# Autodesk Inventor assembly: zitvlak
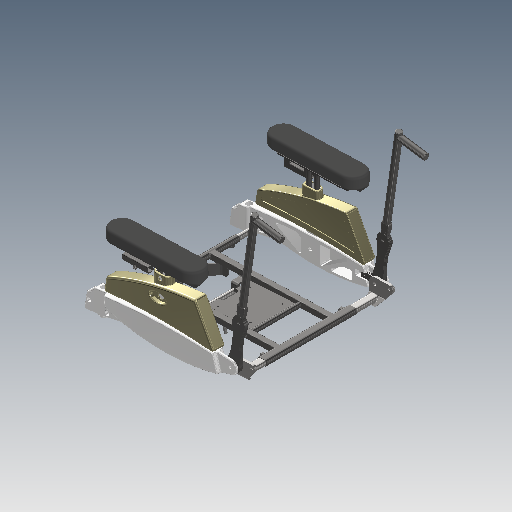
[picture p0: Inventor's stored thumbnail of the model, 512x512]
Saved by Autodesk Inventor 2020.3 (Build 243373000, 373)
## iProperties
Created: 2020-09-15
Part Number: zitvlak
Document SubType Name: Assembly
Designer: Svend
Author: Svend
## Documents named in this file (14)
- C:\Users\Svend\OneDrive\Documents\GitHub\Rolstoel\zitvlak.iam
- C:\Users\Svend\OneDrive\Documents\GitHub\Rolstoel\buis 18 mm.ipt
- C:\Users\Svend\OneDrive\Documents\GitHub\Rolstoel\frame achterkant links.ipt
- C:\Users\Svend\OneDrive\Documents\GitHub\Rolstoel\frame achterkant.ipt
- C:\Users\Svend\OneDrive\Documents\GitHub\Rolstoel\frame zitvlak.ipt
- C:\Users\Svend\OneDrive\Documents\GitHub\Rolstoel\scharnier.iam
- C:\Users\Svend\OneDrive\Documents\GitHub\Rolstoel\stelbuis.ipt
- C:\Users\Svend\OneDrive\Documents\GitHub\Rolstoel\lift connectie.ipt
- C:\Users\Svend\OneDrive\Documents\GitHub\Rolstoel\stelblokje.ipt
- C:\Users\Svend\OneDrive\Documents\GitHub\Rolstoel\zijkant.ipt
- C:\Users\Svend\OneDrive\Documents\GitHub\Rolstoel\armsteun links.iam
- C:\Users\Svend\OneDrive\Documents\GitHub\Rolstoel\zijkant rechts.ipt
- C:\Users\Svend\OneDrive\Documents\GitHub\Rolstoel\armsteun rechts.iam
- C:\Users\Svend\OneDrive\Documents\GitHub\Rolstoel\handvaten.ipt
## Components (16 placed, 13 different names)
1. buis 18 mm:1 — Mate:3, Flush:1, Mate:19
2. frame achterkant links:1 — Mate:2, Angle:2, Mate:5, Mate:6, Angle:3, Mate:8
3. frame achterkant:1 — Mate:1, Angle:1, Mate:7, Mate:9, Mate:10
4. frame zitvlak:1 — Mate:1, Angle:1, Mate:2, Angle:2, Mate:3, Flush:1, Mate:4, Flush:2, Mate:7, Mate:8, Mate:11, Mate:12, Mate:13, Mate:14, Flush:4, Flush:5, Angle:5, Angle:6
5. scharnier:1 [sub-assembly] — Mate:5, Mate:6, Angle:3, Flush:3, Mate:17, Mate:18, Mate:28, Mate:29, Angle:6, Angle:7
6. buis 18 mm:2 — Mate:4, Flush:2, Mate:23
7. scharnier:2 [sub-assembly] — Mate:9, Mate:10, Flush:3, Mate:22, Mate:24, Mate:30, Mate:31
8. stelbuis:1 — Mate:11, Mate:12, Mate:16
9. lift connectie:1 — Mate:13, Mate:14, Mate:15, Angle:5
10. stelblokje:1 — Mate:15, Mate:16
11. zijkant:1 — Mate:17, Mate:18, Mate:19, Flush:4, Flush:5, Mate:20, Mate:21, Mate:32
12. armsteun links:1 [sub-assembly] — Mate:20, Mate:21, Flush:6, Mate:32
13. zijkant rechts:1 — Mate:22, Mate:23, Mate:24, Mate:25, Mate:26
14. armsteun rechts:1 [sub-assembly] — Mate:25, Mate:26, Flush:6
15. handvaten:1 — Mate:28, Mate:29, Flush:7, Angle:7
16. handvaten:2 — Mate:30, Mate:31, Flush:7
## Relationships (44: Mate 31, Flush 7, Angle 6)
- Mate:1: frame achterkant:1 ↔ frame zitvlak:1
- Angle:1 (0 deg): frame achterkant:1 ↔ frame zitvlak:1
- Mate:2: frame achterkant links:1 ↔ frame zitvlak:1
- Angle:2 (0 deg): frame achterkant links:1 ↔ frame zitvlak:1
- Mate:3: buis 18 mm:1 ↔ frame zitvlak:1
- Flush:1 (-55 mm): buis 18 mm:1 ↔ frame zitvlak:1
- Mate:4: frame zitvlak:1 ↔ buis 18 mm:2
- Flush:2 (-55 mm): frame zitvlak:1 ↔ buis 18 mm:2
- Mate:5: frame achterkant links:1 ↔ scharnier:1
- Mate:6: frame achterkant links:1 ↔ scharnier:1
- Angle:3 (0 deg): frame achterkant links:1 ↔ scharnier:1
- Mate:7 (80 mm): frame achterkant:1 ↔ frame zitvlak:1
- Mate:8 (80 mm): frame achterkant links:1 ↔ frame zitvlak:1
- Mate:9: frame achterkant:1 ↔ scharnier:2
- Mate:10: frame achterkant:1 ↔ scharnier:2
- Flush:3: scharnier:1 ↔ scharnier:2
- Mate:11: frame zitvlak:1 ↔ stelbuis:1
- Mate:12: frame zitvlak:1 ↔ stelbuis:1
- Mate:13: frame zitvlak:1 ↔ lift connectie:1
- Mate:14: frame zitvlak:1 ↔ lift connectie:1
- Mate:15: lift connectie:1 ↔ stelblokje:1
- Mate:16: stelbuis:1 ↔ stelblokje:1
- Mate:17: scharnier:1 ↔ zijkant:1
- Mate:18: scharnier:1 ↔ zijkant:1
- Mate:19: buis 18 mm:1 ↔ zijkant:1
- Flush:4: frame zitvlak:1 ↔ zijkant:1
- Flush:5: frame zitvlak:1 ↔ zijkant:1
- Mate:20: zijkant:1 ↔ armsteun links:1
- Mate:21: zijkant:1 ↔ armsteun links:1
- Mate:22: scharnier:2 ↔ zijkant rechts:1
- Mate:23: buis 18 mm:2 ↔ zijkant rechts:1
- Mate:24: scharnier:2 ↔ zijkant rechts:1
- Mate:25: zijkant rechts:1 ↔ armsteun rechts:1
- Mate:26: zijkant rechts:1 ↔ armsteun rechts:1
- Flush:6: armsteun links:1 ↔ armsteun rechts:1
- Mate:28: scharnier:1 ↔ handvaten:1
- Mate:29: scharnier:1 ↔ handvaten:1
- Mate:30: scharnier:2 ↔ handvaten:2
- Mate:31: scharnier:2 ↔ handvaten:2
- Flush:7: handvaten:1 ↔ handvaten:2
- Angle:5 (2 deg): frame zitvlak:1 ↔ lift connectie:1
- Mate:32 (-690 mm): zijkant:1 ↔ armsteun links:1
- Angle:6 (100 deg): frame zitvlak:1 ↔ scharnier:1
- Angle:7 (90 deg): scharnier:1 ↔ handvaten:1
